# Autodesk Inventor assembly: chumacera de 20 mm
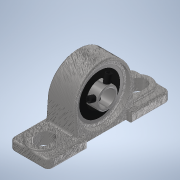
[picture p0: Inventor's stored thumbnail of the model, 180x180]
Saved by Autodesk Inventor 2021 (Build 250183000, 183)
## iProperties
Created: 2012-06-12
Part Number: chumacera de 20 mm
Document SubType Name: Assembly
Designer: Luis
Author: Luis
## Documents named in this file (5)
- C:\Users\79449\Documents\CNC_DISENO_DE MAQUINAS\Piezas-Ensambles_Inventor\Primera_presentación\Chumacera\chumacera de 20 mm.iam
- C:\Users\79449\Documents\CNC_DISENO_DE MAQUINAS\Piezas-Ensambles_Inventor\Primera_presentación\Chumacera\1.ipt
- C:\Users\79449\Documents\CNC_DISENO_DE MAQUINAS\Piezas-Ensambles_Inventor\Primera_presentación\Chumacera\2.ipt
- C:\Users\79449\Documents\CNC_DISENO_DE MAQUINAS\Piezas-Ensambles_Inventor\Primera_presentación\Chumacera\3.ipt
- C:\Users\79449\Documents\CNC_DISENO_DE MAQUINAS\Piezas-Ensambles_Inventor\Primera_presentación\Chumacera\4.ipt
## Components (5 placed, 4 different names)
1. 1:1 — Insert:1
2. 2:1 — Insert:1, Insert:2, Mate:1, Mate:2
3. 3:1 — Insert:2
4. 4:1 — Mate:2
5. 4:2 — Mate:1
## Relationships (4: Insert 2, Mate 2)
- Insert:1: 1:1 ↔ 2:1
- Insert:2: 2:1 ↔ 3:1
- Mate:1: 2:1 ↔ 4:2
- Mate:2: 2:1 ↔ 4:1
